# Autodesk Inventor assembly: Zusammenbau
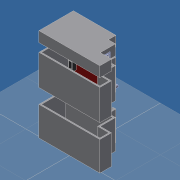
[picture p0: Inventor's stored thumbnail of the model, 180x180]
Saved by Autodesk Inventor 2016 SP2 (Build 200236200, 236)
## iProperties
Created: 2018-07-08
Part Number: Zusammenbau
Material: Generisch
Document SubType Name: Assembly
Designer: User
Author: User
## Documents named in this file (6)
- C:\Users\User\Documents\Inventor\Hutschinengehäuse\Zusammenbau.iam
- C:\Users\User\Documents\Inventor\Hutschinengehäuse\ReprapDiscountFullGraphicSmartController-Robotale_Dummy.ipt
- C:\Users\User\Documents\Inventor\Hutschinengehäuse\ArduinoMega.ipt
- C:\Users\User\Documents\Inventor\Hutschinengehäuse\Basis.ipt
- C:\Users\User\Documents\Inventor\Hutschinengehäuse\Display.ipt
- C:\Users\User\Documents\Inventor\Hutschinengehäuse\Erweiterung.ipt
## Components (5 placed, 5 different names)
1. ReprapDiscountFullGraphicSmartController-Robotale_Dummy:1 — Passend:9, Passend:10, Passend:11, Passend:12, Passend:14
2. ArduinoMega:1 — Passend:6, Passend:7, Passend:8
3. Basis:1 — Passend:6, Passend:7, Passend:8, Passend:9, Passend:10
4. Display:1 — Passend:11, Passend:12, Fluchtend:14
5. Erweiterung:1 — Fluchtend:14, Passend:14
## Relationships (9: Mate 8, Flush 1)
- Passend:6 [Mate]: ArduinoMega:1 ↔ Basis:1
- Passend:7 [Mate]: ArduinoMega:1 ↔ Basis:1
- Passend:8 [Mate]: ArduinoMega:1 ↔ Basis:1
- Passend:9 [Mate]: ReprapDiscountFullGraphicSmartController-Robotale_Dummy:1 ↔ Basis:1
- Passend:10 [Mate]: ReprapDiscountFullGraphicSmartController-Robotale_Dummy:1 ↔ Basis:1
- Passend:11 [Mate]: ReprapDiscountFullGraphicSmartController-Robotale_Dummy:1 ↔ Display:1
- Passend:12 [Mate]: ReprapDiscountFullGraphicSmartController-Robotale_Dummy:1 ↔ Display:1
- Fluchtend:14 [Flush]: Display:1 ↔ Erweiterung:1
- Passend:14 [Mate]: ReprapDiscountFullGraphicSmartController-Robotale_Dummy:1 ↔ Erweiterung:1
